# Autodesk Inventor assembly: Front Hub Carrier L new
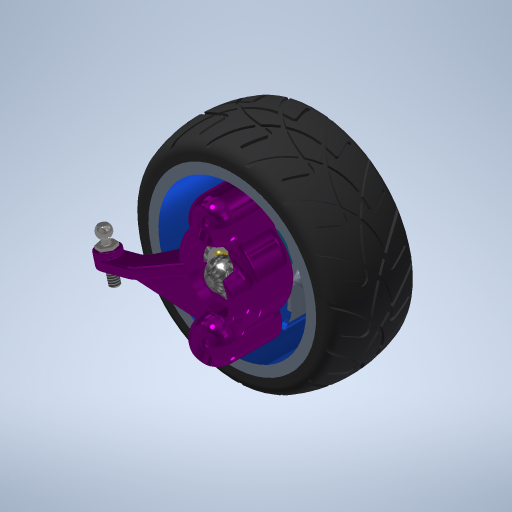
[picture p0: Inventor's stored thumbnail of the model, 512x512]
Saved by Autodesk Inventor 2023 (Build 270158000, 158)
## iProperties
Created: 2019-12-03
Part Number: Front Hub Carrier L new
Document SubType Name: Assembly
Designer: Jopa
Author: Jopa
## Documents named in this file (12)
- C:\Users\CASPER\Desktop\HUDSON süspansiyon\Front Hub Carrier L new.iam
- C:\Users\CASPER\Desktop\HUDSON süspansiyon\Front Hub Carrier L.ipt
- C:\Users\CASPER\Desktop\HUDSON süspansiyon\Pillow Ball Retainer.ipt
- C:\Users\CASPER\Desktop\HUDSON süspansiyon\Pillow Ball Bushing.ipt
- C:\Users\CASPER\Desktop\HUDSON süspansiyon\Pillow Ball Retainer_CPY.ipt
- C:\Users\CASPER\Desktop\HUDSON süspansiyon\Pillow Ball Bushing_CPY.ipt
- C:\Users\CASPER\Desktop\HUDSON süspansiyon\Front Axel.ipt
- C:\Users\CASPER\Desktop\HUDSON süspansiyon\0.1875 Ball Stud 0.375.ipt
- C:\Users\CASPER\Desktop\HUDSON süspansiyon\Rear Hex Hub.iam
- C:\Users\CASPER\Desktop\HUDSON süspansiyon\Wheel L.iam
- C:\Users\CASPER\Desktop\HUDSON süspansiyon\ANSI B18.2.4.4M - M5 x 0,8.ipt
- C:\Users\CASPER\Desktop\HUDSON süspansiyon\Assemblybearing.iam
## Components (12 placed, 11 different names)
1. Front Hub Carrier L:1 — Mate:3, Mate:4, Mate:7, Mate:8, Mate:9, Insert:3, Mate:18, Mate:19, Mate:20, Mate:21
2. Pillow Ball Retainer:1 — Mate:1, Mate:2, Mate:3
3. Pillow Ball Bushing:1 — Mate:1, Mate:2, Mate:4
4. Pillow Ball Retainer_CPY:1 — Mate:5, Mate:6, Mate:8
5. Pillow Ball Bushing_CPY:1 — Mate:5, Mate:6, Mate:7
6. Front Axel:1 — Mate:9, Mate:11, Mate:12, Mate:13, Mate:16
7. 0.1875 Ball Stud 0.375:1 — Insert:3
8. Rear Hex Hub:1 [sub-assembly] — Mate:11, Mate:12, Mate:14, Mate:15
9. Wheel L:1 [sub-assembly] — Mate:13, Mate:14, Mate:15, Mate:17
10. ANSI B18.2.4.4M - M5 x 0,8:1 — Mate:16, Mate:17
11. Assemblybearing:1 [sub-assembly] — Mate:18, Mate:19
12. Assemblybearing:2 [sub-assembly] — Mate:20, Mate:21
## Relationships (21: Mate 20, Insert 1)
- Mate:1: Pillow Ball Retainer:1 ↔ Pillow Ball Bushing:1
- Mate:2: Pillow Ball Retainer:1 ↔ Pillow Ball Bushing:1
- Mate:3: Front Hub Carrier L:1 ↔ Pillow Ball Retainer:1
- Mate:4: Front Hub Carrier L:1 ↔ Pillow Ball Bushing:1
- Mate:5: Pillow Ball Retainer_CPY:1 ↔ Pillow Ball Bushing_CPY:1
- Mate:6: Pillow Ball Retainer_CPY:1 ↔ Pillow Ball Bushing_CPY:1
- Mate:7: Front Hub Carrier L:1 ↔ Pillow Ball Bushing_CPY:1
- Mate:8: Front Hub Carrier L:1 ↔ Pillow Ball Retainer_CPY:1
- Mate:9: Front Hub Carrier L:1 ↔ Front Axel:1
- Insert:3: Front Hub Carrier L:1 ↔ 0.1875 Ball Stud 0.375:1
- Mate:11: Front Axel:1 ↔ Rear Hex Hub:1
- Mate:12: Front Axel:1 ↔ Rear Hex Hub:1
- Mate:13: Front Axel:1 ↔ Wheel L:1
- Mate:14: Rear Hex Hub:1 ↔ Wheel L:1
- Mate:15: Rear Hex Hub:1 ↔ Wheel L:1
- Mate:16: Front Axel:1 ↔ ANSI B18.2.4.4M - M5 x 0,8:1
- Mate:17: Wheel L:1 ↔ ANSI B18.2.4.4M - M5 x 0,8:1
- Mate:18: Front Hub Carrier L:1 ↔ Assemblybearing:1
- Mate:19: Front Hub Carrier L:1 ↔ Assemblybearing:1
- Mate:20: Front Hub Carrier L:1 ↔ Assemblybearing:2
- Mate:21: Front Hub Carrier L:1 ↔ Assemblybearing:2
